# Autodesk Inventor assembly: Super Gantry
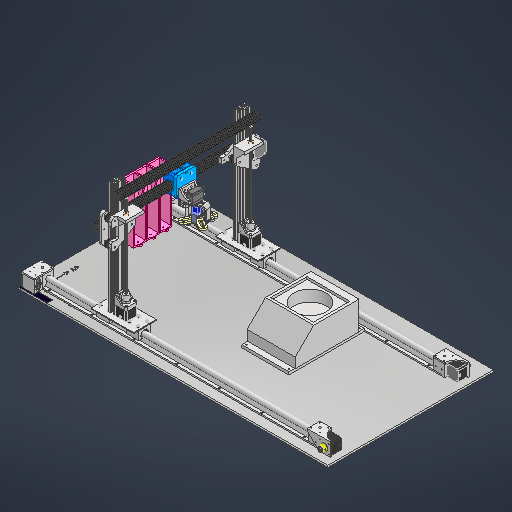
[picture p0: Inventor's stored thumbnail of the model, 512x512]
Saved by Autodesk Inventor 2025.1 (Build 291241000, 241)
## iProperties
Created: 2025-01-22
Part Number: Super Gantry
Document SubType Name: Assembly
Designer: jerem
Author: jerem
## Documents named in this file (11)
- C:\Users\jerem\Documents\GitHub\Perovskite-Automated-Synthesis-System\CAD\Gantry\Super Gantry.iam
- C:\Users\jerem\Documents\GitHub\Perovskite-Automated-Synthesis-System\CAD\Gantry\X Axis.iam
- C:\Users\jerem\Documents\GitHub\Perovskite-Automated-Synthesis-System\CAD\Gantry\Z Axis.iam
- C:\Users\jerem\Documents\GitHub\Perovskite-Automated-Synthesis-System\CAD\Toolhead\Toolhead.iam
- C:\Users\jerem\Documents\GitHub\Perovskite-Automated-Synthesis-System\CAD\Camera\Camera Assembly.iam
- C:\Users\jerem\Documents\GitHub\Perovskite-Automated-Synthesis-System\CAD\Gripper\Redesign_GripperASSEM.iam
- C:\Users\jerem\Documents\GitHub\Perovskite-Automated-Synthesis-System\CAD\Non 3D Printed Parts\Spin Coater.ipt
- C:\Users\jerem\Documents\GitHub\Perovskite-Automated-Synthesis-System\CAD\Object Mounts\Spincoater Base Mount.ipt
- C:\Users\jerem\Documents\GitHub\Perovskite-Automated-Synthesis-System\CAD\Gantry\Y Axis.iam
- C:\Users\jerem\Documents\GitHub\Perovskite-Automated-Synthesis-System\CAD\Pipette\PipetteStand.ipt
- C:\Users\jerem\Documents\GitHub\Perovskite-Automated-Synthesis-System\CAD\Non 3D Printed Parts\Extrusion\V Extrustion 20x500mm.ipt
## Components (13 placed, 10 different names)
1. X Axis:1 [sub-assembly] — Mate:17, Mate:25, Mate:26, Mate:27, Mate:33, Mate:34
2. Z Axis:1 [sub-assembly] — Flush:4, Flush:5, Mate:34, Mate:37, Mate:39, Flush:6, Mate:40
3. Z Axis:2 [sub-assembly] — Flush:4, Flush:5, Mate:33, Mate:38
4. Toolhead:1 [sub-assembly] — Mate:8, Mate:9, Mate:10, Mate:11, Mate:12, Mate:13, Flush:1, Angle:1, Mate:36
5. Camera Assembly:1 [sub-assembly] — Mate:8, Mate:9, Mate:10
6. Redesign_GripperASSEM:1 [sub-assembly] — Mate:11, Mate:12, Mate:13
7. Spin Coater:1 — Mate:14, Mate:15, Mate:16
8. Spincoater Base Mount:1 — Mate:14, Mate:15, Mate:16, Mate:17
9. Y Axis:1 [sub-assembly] — Flush:1, Angle:1, Mate:36, Mate:37, Mate:38
10. PipetteStand:1 — Mate:26, Mate:28, Mate:29, Flush:2
11. PipetteStand:2 — Mate:25, Mate:28, Flush:2, Flush:3
12. PipetteStand:3 — Mate:27, Mate:29, Flush:3
13. V Extrustion 20x500mm:1 — Mate:39, Flush:6, Mate:40
## Relationships (29: Mate 22, Flush 6, Angle 1)
- Mate:8: Toolhead:1 ↔ Camera Assembly:1
- Mate:9: Toolhead:1 ↔ Camera Assembly:1
- Mate:10: Toolhead:1 ↔ Camera Assembly:1
- Mate:11: Toolhead:1 ↔ Redesign_GripperASSEM:1
- Mate:12: Toolhead:1 ↔ Redesign_GripperASSEM:1
- Mate:13: Toolhead:1 ↔ Redesign_GripperASSEM:1
- Mate:14: Spin Coater:1 ↔ Spincoater Base Mount:1
- Mate:15: Spin Coater:1 ↔ Spincoater Base Mount:1
- Mate:16: Spin Coater:1 ↔ Spincoater Base Mount:1
- Mate:17: X Axis:1 ↔ Spincoater Base Mount:1
- Flush:1: Toolhead:1 ↔ Y Axis:1
- Mate:25: X Axis:1 ↔ PipetteStand:2
- Mate:26: X Axis:1 ↔ PipetteStand:1
- Mate:27: X Axis:1 ↔ PipetteStand:3
- Mate:28: PipetteStand:1 ↔ PipetteStand:2
- Mate:29: PipetteStand:1 ↔ PipetteStand:3
- Flush:2: PipetteStand:1 ↔ PipetteStand:2
- Flush:3: PipetteStand:2 ↔ PipetteStand:3
- Flush:4: Z Axis:1 ↔ Z Axis:2
- Flush:5: Z Axis:1 ↔ Z Axis:2
- Angle:1 (180 deg): Toolhead:1 ↔ Y Axis:1
- Mate:36: Toolhead:1 ↔ Y Axis:1
- Mate:33: X Axis:1 ↔ Z Axis:2
- Mate:34: X Axis:1 ↔ Z Axis:1
- Mate:37: Z Axis:1 ↔ Y Axis:1
- Mate:38: Z Axis:2 ↔ Y Axis:1
- Mate:39: Z Axis:1 ↔ V Extrustion 20x500mm:1
- Flush:6: Z Axis:1 ↔ V Extrustion 20x500mm:1
- Mate:40: Z Axis:1 ↔ V Extrustion 20x500mm:1
